# Autodesk Inventor assembly: Ensamblaje1
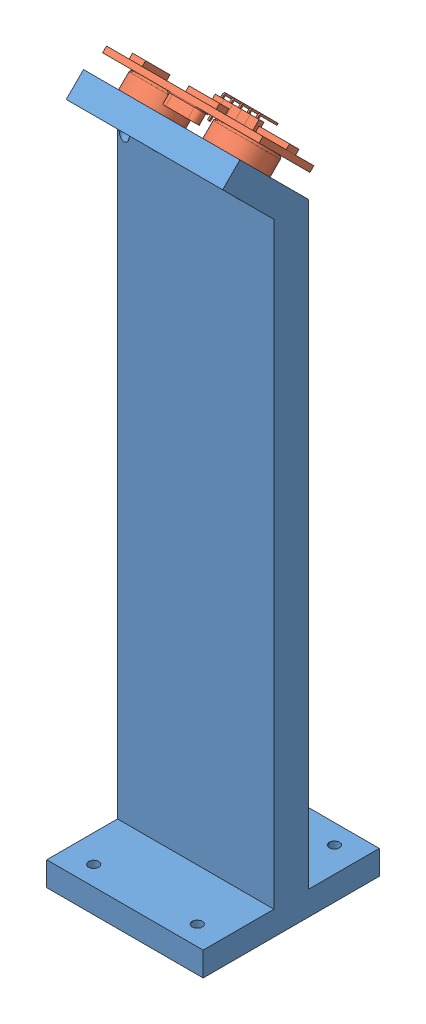
[picture p0: shaded view drawn from the part files that the assembly names]
Saved by Autodesk Inventor 2026 (Build 300175000, 175)
## iProperties
Created: 2025-06-27
Part Number: Ensamblaje1
Document SubType Name: Assembly
Designer: oscar
Author: oscar
## Documents named in this file (3)
- C:\Users\oscar\Downloads\SmartChef\CAD\Ensamblaje1.iam
- C:\Users\oscar\Downloads\SmartChef\CAD\Soporte_Ultrasonido.ipt
- C:\Users\oscar\Downloads\SmartChef\CAD\hy-srf05-ultrasonic-1.snapshot.5\HY-SRF05\HY-SRF05\HY-SRF05\HY-SRF05.ipt
## Components (2 placed, 2 different names)
1. Soporte_Ultrasonido:1 — Rígido:1
2. HY-SRF05:1 — Rígido:1
## Relationships (1: WeldJoint 1)
- Rígido:1 [WeldJoint]: Soporte_Ultrasonido:1 ↔ HY-SRF05:1
